# Autodesk Inventor assembly: Unit_SR-I
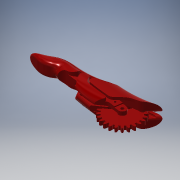
[picture p0: Inventor's stored thumbnail of the model, 180x180]
Saved by Autodesk Inventor 2018.2 (Build 222227000, 227)
## iProperties
Created: 2018-02-15
Part Number: Unit_SR-I
Material: 一般
Document SubType Name: Assembly
Designer: sktom
Author: sktom
Title: Unit_SR-I
## Documents named in this file (11)
- D:\CloudStrage\OneDrive\CADMech\HbSizeSMech\UnitHand\Unit_SR-H\Unit_SR-I\Unit_SR-I.iam
- D:\CloudStrage\OneDrive\CADMech\HbSizeSMech\UnitHand\Unit_SR-H\Unit_SR-I\SR-I-03.ipt
- D:\CloudStrage\OneDrive\CADMech\HbSizeSMech\UnitHand\Unit_SR-H\Unit_SR-I\SR-I-02.ipt
- D:\CloudStrage\OneDrive\CADMech\HbSizeSMech\UnitHand\Unit_SR-H\Unit_SR-I\SR-I-04.ipt
- D:\CloudStrage\OneDrive\CADMech\HbSizeSMech\UnitHand\Unit_SR-H\Unit_SR-I\SR-I-01.ipt
- D:\CloudStrage\OneDrive\CADMech\HbSizeSMech\UnitHand\Unit_SR-H\Unit_SR-I\SR-I-05.ipt
- D:\CloudStrage\OneDrive\CADMech\HbSizeSMech\UnitHand\Unit_SR-H\Unit_SR-I\SR-I-06.ipt
- D:\CloudStrage\OneDrive\CADMech\HbSizeSMech\UnitHand\Unit_SR-H\Unit_SR-I\SR-I-07.ipt
- D:\CloudStrage\OneDrive\CADMech\HbSizeSMech\UnitHand\Unit_SR-H\Unit_SR-I\Parts_Screw_M1.4_L6.ipt
- D:\CloudStrage\OneDrive\CADMech\HbSizeSMech\UnitHand\Unit_SR-H\Unit_SR-I\Parts_Shaft_Phi1.5_L6.ipt
- D:\CloudStrage\OneDrive\CADMech\HbSizeSMech\UnitHand\Unit_SR-H\Unit_SR-I\Parts_TOS 0.3-3-270ﾟ-3.ipt
## Components (16 placed, 10 different names)
1. SR-I-01 — 挿入:4, 挿入:7, 回転:1, 回転:2
2. SR-I-02 — 挿入:1, 挿入:2, 挿入:3, 挿入:4, 挿入:9, 挿入:10
3. SR-I-03 — 挿入:3, 円柱状:1, 回転:4
4. SR-I-04 — 挿入:1, 挿入:2
5. SR-I-05 — 挿入:8, 回転:3
6. SR-I-06 — 挿入:5, 挿入:6, 挿入:7, 円柱状:1, 挿入:8, 挿入:11, 挿入:12
7. SR-I-07 — 挿入:5, 挿入:6
8. Parts_Screw_M1.4_L6:1 — 挿入:12
9. Parts_Screw_M1.4_L6:2 — 挿入:11
10. Parts_Screw_M1.4_L6:3 — 挿入:10
11. Parts_Screw_M1.4_L6:4 — 挿入:9
12. Parts_Shaft_Phi1.5_L6:1 — 回転:1
13. Parts_Shaft_Phi1.5_L6:2 — 回転:2
14. Parts_Shaft_Phi1.5_L6:3 — 回転:4
15. Parts_Shaft_Phi1.5_L6:4 — 回転:3
16. Parts_TOS 0.3-3-270ﾟ-3:1
## Relationships (17: Insert 12, RevoluteJoint 4, CylindricalJoint 1)
- 挿入:1 [Insert]: SR-I-02 ↔ SR-I-04
- 挿入:2 [Insert]: SR-I-02 ↔ SR-I-04
- 挿入:3 [Insert] (0.107 mm): SR-I-02 ↔ SR-I-03
- 挿入:4 [Insert] (0.145 mm): SR-I-01 ↔ SR-I-02
- 挿入:5 [Insert]: SR-I-06 ↔ SR-I-07
- 挿入:6 [Insert]: SR-I-06 ↔ SR-I-07
- 挿入:7 [Insert] (0.026 mm): SR-I-01 ↔ SR-I-06
- 円柱状:1 [CylindricalJoint]: SR-I-03 ↔ SR-I-06
- 挿入:8 [Insert] (0.38 mm): SR-I-05 ↔ SR-I-06
- 挿入:9 [Insert]: SR-I-02 ↔ Parts_Screw_M1.4_L6:4
- 挿入:10 [Insert]: SR-I-02 ↔ Parts_Screw_M1.4_L6:3
- 挿入:11 [Insert]: SR-I-06 ↔ Parts_Screw_M1.4_L6:2
- 挿入:12 [Insert]: SR-I-06 ↔ Parts_Screw_M1.4_L6:1
- 回転:1 [RevoluteJoint] (0.725 mm): SR-I-01 ↔ Parts_Shaft_Phi1.5_L6:1
- 回転:2 [RevoluteJoint] (0.725 mm): SR-I-01 ↔ Parts_Shaft_Phi1.5_L6:2
- 回転:3 [RevoluteJoint]: SR-I-05 ↔ Parts_Shaft_Phi1.5_L6:4
- 回転:4 [RevoluteJoint]: SR-I-03 ↔ Parts_Shaft_Phi1.5_L6:3
